# Autodesk Inventor assembly: Assembly1
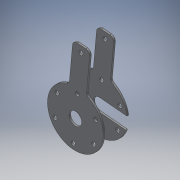
[picture p0: Inventor's stored thumbnail of the model, 180x180]
Saved by Autodesk Inventor 2016 (Build 200138000, 138)
## iProperties
Created: 2015-07-20
Part Number: Assembly1
Document SubType Name: Assembly
Designer: chdsbd
Author: chdsbd
## Documents named in this file (3)
- C:\Users\chdsbd\Dropbox\Assembly1.iam
- C:\Users\chdsbd\Desktop\door_clamp.ipt
- C:\Users\chdsbd\Desktop\door_clamp_back.ipt
## Components (2 placed, 2 different names)
1. door_clamp:1 — Mate:1, Mate:3
2. door_clamp_back:1 — Mate:1, Mate:3
## Relationships (2: Mate 2)
- Mate:1: door_clamp:1 ↔ door_clamp_back:1
- Mate:3: door_clamp:1 ↔ door_clamp_back:1
